# Autodesk Inventor assembly: Air ventilator
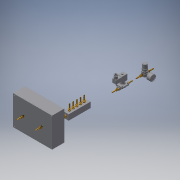
[picture p0: Inventor's stored thumbnail of the model, 180x180]
Saved by Autodesk Inventor 2018 (Build 220112000, 112)
## iProperties
Created: 2020-03-28
Part Number: Air ventilator
Document SubType Name: Assembly
Designer: emile
Author: emile
## Documents named in this file (8)
- C:\Users\emile\OneDrive\Documents\Inventor\Respirator\Peep\AirPressure\Air ventilator.iam
- C:\Users\emile\OneDrive\Documents\Inventor\Respirator\Peep\AirPressure\4711K513_BRASS SOLENOID VALVE.ipt
- C:\Users\emile\OneDrive\Documents\Inventor\Respirator\Peep\AirPressure\Brass Barbed Hose Fitting for Air and Water.ipt
- C:\Users\emile\OneDrive\Documents\Inventor\Respirator\Peep\AirPressure\AR2000 G1-4in Air Control Compressor Pressure Gauge Regulator Relief.ipt
- C:\Users\emile\OneDrive\Documents\Inventor\Respirator\Peep\AirPressure\CorollaAirFilterCase.ipt
- C:\Users\emile\OneDrive\Documents\Inventor\Respirator\Peep\AirPressure\CorollaAirFilter.ipt
- C:\Users\emile\OneDrive\Documents\Inventor\Respirator\Peep\AirPressure\CorollaAirFilterCaseCover.ipt
- C:\Users\emile\OneDrive\Documents\Inventor\Respirator\Peep\AirPressure\Splitter.ipt
## Components (19 placed, 7 different names)
1. 4711K513_BRASS SOLENOID VALVE:1 — Mate:1, Mate:2, Mate:3, Mate:4, Flush:1, Flush:2
2. Brass Barbed Hose Fitting for Air and Water:1 — Mate:1, Mate:4, Mate:9, Mate:10
3. Brass Barbed Hose Fitting for Air and Water:2 — Mate:2, Mate:3
4. AR2000 G1-4in Air Control Compressor Pressure Gauge Regulator Relief:1 — Mate:5, Mate:6, Mate:7, Mate:8, Angle:1, Mate:11
5. Brass Barbed Hose Fitting for Air and Water:3 — Mate:5, Mate:8, Mate:9
6. Brass Barbed Hose Fitting for Air and Water:4 — Mate:6, Mate:7, Mate:10
7. CorollaAirFilterCase:1 — Mate:12, Flush:3, Mate:13, Mate:14, Mate:15, Mate:20, Mate:21, Mate:22, Mate:23
8. CorollaAirFilter:1 — Mate:12, Flush:3, Mate:13, Flush:4
9. CorollaAirFilterCaseCover:1 — Mate:14, Flush:4, Mate:15, Mate:16, Mate:17, Mate:18, Mate:19
10. Brass Barbed Hose Fitting for Air and Water:5 — Mate:16, Mate:17
11. Brass Barbed Hose Fitting for Air and Water:6 — Mate:18, Mate:19
12. Brass Barbed Hose Fitting for Air and Water:7 — Mate:20, Mate:21
13. Splitter:1 — Mate:24, Mate:25, Mate:26, Mate:27, Mate:28, Mate:29
14. Brass Barbed Hose Fitting for Air and Water:8 — Mate:26, Mate:27
15. Brass Barbed Hose Fitting for Air and Water:9 — Mate:28, Mate:29
16. Brass Barbed Hose Fitting for Air and Water:10
17. Brass Barbed Hose Fitting for Air and Water:11
18. Brass Barbed Hose Fitting for Air and Water:12
19. Brass Barbed Hose Fitting for Air and Water:13
## Component patterns: (5 elements, first: Brass Barbed Hose Fitting for Air and Water:9)
## Relationships (34: Mate 29, Flush 4, Angle 1)
- Mate:1: 4711K513_BRASS SOLENOID VALVE:1 ↔ Brass Barbed Hose Fitting for Air and Water:1
- Mate:2: 4711K513_BRASS SOLENOID VALVE:1 ↔ Brass Barbed Hose Fitting for Air and Water:2
- Mate:3: 4711K513_BRASS SOLENOID VALVE:1 ↔ Brass Barbed Hose Fitting for Air and Water:2
- Mate:4: 4711K513_BRASS SOLENOID VALVE:1 ↔ Brass Barbed Hose Fitting for Air and Water:1
- Mate:5: AR2000 G1-4in Air Control Compressor Pressure Gauge Regulator Relief:1 ↔ Brass Barbed Hose Fitting for Air and Water:3
- Mate:6: AR2000 G1-4in Air Control Compressor Pressure Gauge Regulator Relief:1 ↔ Brass Barbed Hose Fitting for Air and Water:4
- Mate:7: AR2000 G1-4in Air Control Compressor Pressure Gauge Regulator Relief:1 ↔ Brass Barbed Hose Fitting for Air and Water:4
- Mate:8: AR2000 G1-4in Air Control Compressor Pressure Gauge Regulator Relief:1 ↔ Brass Barbed Hose Fitting for Air and Water:3
- Mate:9: Brass Barbed Hose Fitting for Air and Water:1 ↔ Brass Barbed Hose Fitting for Air and Water:3
- Mate:10 (25.4 mm): Brass Barbed Hose Fitting for Air and Water:1 ↔ Brass Barbed Hose Fitting for Air and Water:4
- Flush:1: 4711K513_BRASS SOLENOID VALVE:1
- Angle:1 (0 deg): AR2000 G1-4in Air Control Compressor Pressure Gauge Regulator Relief:1
- Flush:2: 4711K513_BRASS SOLENOID VALVE:1
- Mate:11: AR2000 G1-4in Air Control Compressor Pressure Gauge Regulator Relief:1
- Mate:12: CorollaAirFilterCase:1 ↔ CorollaAirFilter:1
- Flush:3: CorollaAirFilterCase:1 ↔ CorollaAirFilter:1
- Mate:13: CorollaAirFilterCase:1 ↔ CorollaAirFilter:1
- Mate:14: CorollaAirFilterCase:1 ↔ CorollaAirFilterCaseCover:1
- Flush:4: CorollaAirFilter:1 ↔ CorollaAirFilterCaseCover:1
- Mate:15: CorollaAirFilterCase:1 ↔ CorollaAirFilterCaseCover:1
- Mate:16: CorollaAirFilterCaseCover:1 ↔ Brass Barbed Hose Fitting for Air and Water:5
- Mate:17: CorollaAirFilterCaseCover:1 ↔ Brass Barbed Hose Fitting for Air and Water:5
- Mate:18: CorollaAirFilterCaseCover:1 ↔ Brass Barbed Hose Fitting for Air and Water:6
- Mate:19: CorollaAirFilterCaseCover:1 ↔ Brass Barbed Hose Fitting for Air and Water:6
- Mate:20: CorollaAirFilterCase:1 ↔ Brass Barbed Hose Fitting for Air and Water:7
- Mate:21: CorollaAirFilterCase:1 ↔ Brass Barbed Hose Fitting for Air and Water:7
- Mate:22: CorollaAirFilterCase:1
- Mate:23: CorollaAirFilterCase:1
- Mate:24: Splitter:1
- Mate:25: Splitter:1
- Mate:26: Splitter:1 ↔ Brass Barbed Hose Fitting for Air and Water:8
- Mate:27: Splitter:1 ↔ Brass Barbed Hose Fitting for Air and Water:8
- Mate:28: Splitter:1 ↔ Brass Barbed Hose Fitting for Air and Water:9
- Mate:29: Splitter:1 ↔ Brass Barbed Hose Fitting for Air and Water:9
